# Autodesk Inventor assembly: Y Slider
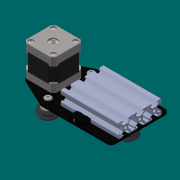
[picture p0: Inventor's stored thumbnail of the model, 180x180]
Saved by Autodesk Inventor 2016 (Build 200138000, 138)
## iProperties
Created: 2015-06-04
Part Number: Y Slider
Document SubType Name: Assembly
Designer: Sawaiz Syed
Author: Sawaiz Syed
## Documents named in this file (7)
- C:\Users\Sawaiz\Documents\data\projects\cncBlackBox\yAxis\ySlider.iam
- C:\Users\Sawaiz\Documents\data\projects\cncBlackBox\yAxis\ySliderPlate.ipt
- C:\Users\Sawaiz\Documents\data\projects\cncBlackBox\nema17Stepper\nema17t5.iam
- C:\Users\Sawaiz\Documents\data\projects\cncBlackBox\vWheel\vWheelSpacer.iam
- C:\Users\Sawaiz\Documents\data\projects\cncBlackBox\yAxis\sliderMountingExtrution.ipt
- C:\Users\Sawaiz\Documents\data\projects\cncBlackBox\vWheel\vWheelEccentricTNut.iam
- C:\Users\Sawaiz\Documents\data\projects\cncBlackBox\microswitch\noLeverMicroswitch.iam
## Components (7 placed, 6 different names)
1. ySliderPlate:1 — Mate:1, Mate:2, Angle:1, Mate:4, Mate:5, Mate:7, Flush:3, Mate:8, Mate:11, Mate:12, Mate:13, Flush:4
2. nema17t5:1 [sub-assembly] — Mate:1, Mate:2, Angle:1
3. vWheelSpacer:1 [sub-assembly] — Mate:4, Flush:1, Mate:12
4. vWheelEccentricTNut:1 [sub-assembly] — Mate:8, Mate:10, Mate:11
5. vWheelSpacer:2 [sub-assembly] — Mate:5, Flush:1
6. sliderMountingExtrution:1 — Mate:7, Flush:3, Mate:10
7. noLeverMicroswitch:1 [sub-assembly] — Mate:13, Flush:4
## Relationships (14: Mate 10, Flush 3, Angle 1)
- Mate:1: ySliderPlate:1 ↔ nema17t5:1
- Mate:2: ySliderPlate:1 ↔ nema17t5:1
- Angle:1 (0 deg): ySliderPlate:1 ↔ nema17t5:1
- Mate:4: ySliderPlate:1 ↔ vWheelSpacer:1
- Mate:5: ySliderPlate:1 ↔ vWheelSpacer:2
- Flush:1: vWheelSpacer:1 ↔ vWheelSpacer:2
- Mate:7: ySliderPlate:1 ↔ sliderMountingExtrution:1
- Flush:3: ySliderPlate:1 ↔ sliderMountingExtrution:1
- Mate:8: ySliderPlate:1 ↔ vWheelEccentricTNut:1
- Mate:10 (0.5 mm): vWheelEccentricTNut:1 ↔ sliderMountingExtrution:1
- Mate:11: ySliderPlate:1 ↔ vWheelEccentricTNut:1
- Mate:12: ySliderPlate:1 ↔ vWheelSpacer:1
- Mate:13: ySliderPlate:1 ↔ noLeverMicroswitch:1
- Flush:4: ySliderPlate:1 ↔ noLeverMicroswitch:1
